# Autodesk Inventor assembly: 3d_Welding_Tooling - Lathe carriage
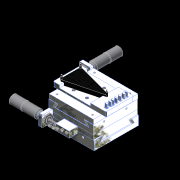
[picture p0: Inventor's stored thumbnail of the model, 180x180]
Saved by Autodesk Inventor 2018.3 (Build 223284000, 284)
## iProperties
Created: 2026-02-27
Part Number: 3d_Welding_Tooling - Lathe carriage
Document SubType Name: Assembly
Designer: aca6
Author: aca6
## Documents named in this file (19)
- C:\Users\aca6\git\LM\items\hw_LM\variants\items\Welding Tooling\3d\3d_Welding_Tooling - Lathe carriage.iam
- C:\Users\aca6\git\LM\items\hw_LM\variants\items\Welding Tooling\3d\3d_Welding_Tooling - Adapter.ipt
- C:\Users\aca6\git\LM\items\hw_LM\variants\items\Welding Tooling\3d\3d_Welding_Tooling -  Guide Pin.ipt
- C:\Users\aca6\git\LM\items\hw_LM\variants\items\Welding Tooling\3d\3d_Welding_Tooling - Top Adapter.ipt
- C:\Users\aca6\git\LM\items\hw_LM\variants\items\Welding Tooling\3d\3d_Welding_Tooling - Moving base.ipt
- C:\Users\aca6\git\LM\items\hw_LM\variants\items\Welding Tooling\3d\3d_Welding_Tooling - Fixed base.ipt
- C:\Users\aca6\git\LM\items\hw_LM\variants\items\Welding Tooling\3d\3d_Welding_Tooling - Acetal Stick.ipt
- C:\Users\aca6\git\LM\items\hw_LM\variants\items\Welding Tooling\3d\3d_Welding_Tooling - Upper fixed base.ipt
- C:\Users\aca6\git\LM\items\hw_LM\variants\items\Welding Tooling\3d\3d_Welding_Tooling - Upper moving base.ipt
- C:\Users\aca6\git\LM\items\_accesories\Tornilleria\Tornillos\3d_DIN 7991\3d\A4 Black Inox\DIN 7991 - M3x14 Black INOX.ipt
- C:\Users\aca6\git\LM\items\_accesories\Tornilleria\Tornillos\3d_DIN 7991\3d\A4 Black Inox\DIN 7991 - M3x12 Black INOX.ipt
- C:\Users\aca6\git\LM\items\hw_LM\variants\items\Welding Tooling\3d\3d_Welding_Tooling -  Micrometer Nut.ipt
- C:\Users\aca6\git\LM\items\hw_LM\variants\items\Welding Tooling\3d\3d_Welding_Tooling -  Micrometer.ipt
- C:\Users\aca6\git\LM\items\hw_LM\variants\items\Welding Tooling\3d\3d_Welding_Tooling - Fixed Block.ipt
- C:\Users\aca6\git\LM\items\hw_LM\variants\items\Welding Tooling\3d\3d_Welding_Tooling -  Moving Block.ipt
- C:\Users\aca6\git\LM\items\_accesories\Tornilleria\Tornillos\3d_Accu Group\3d\Prisionero nylon M4x7 REF SSN-M4-7.ipt
- C:\Users\aca6\git\LM\items\_accesories\Tornilleria\Tornillos\3d_DIN 912\3d\A4 Inox\DIN 912 - M3 x 0,5 x 8 -  INOX.ipt
- C:\Users\aca6\git\LM\items\_accesories\Tornilleria\Tornillos\3d_DIN 912\3d\A4 Inox\DIN 912 - M3 x 0,5 x 30 -  INOX.ipt
- C:\Users\aca6\git\LM\items\_accesories\Tornilleria\Tornillos\3d_DIN 912\3d\A4 Inox\DIN 912 - M3 x 0,5 x 10 -  INOX.ipt
## Components (51 placed, 18 different names)
1. 3d_Welding_Tooling - Adapter:1
2. 3d_Welding_Tooling -  Guide Pin:1
3. 3d_Welding_Tooling -  Guide Pin:2
4. 3d_Welding_Tooling -  Guide Pin:3
5. 3d_Welding_Tooling - Top Adapter:1
6. 3d_Welding_Tooling - Moving base:1
7. 3d_Welding_Tooling - Fixed base:1
8. 3d_Welding_Tooling - Acetal Stick:1
9. 3d_Welding_Tooling - Acetal Stick:2
10. 3d_Welding_Tooling - Upper fixed base:1
11. 3d_Welding_Tooling - Acetal Stick:3
12. 3d_Welding_Tooling - Acetal Stick:4
13. 3d_Welding_Tooling - Upper moving base:1
14. DIN 7991 - M3x14 Black INOX:1
15. DIN 7991 - M3x14 Black INOX:2
16. DIN 7991 - M3x14 Black INOX:3
17. DIN 7991 - M3x14 Black INOX:4
18. DIN 7991 - M3x12 Black INOX:1
19. DIN 7991 - M3x12 Black INOX:2
20. DIN 7991 - M3x12 Black INOX:3
21. DIN 7991 - M3x12 Black INOX:4
22. 3d_Welding_Tooling -  Micrometer Nut:1
23. 3d_Welding_Tooling -  Micrometer:1
24. 3d_Welding_Tooling -  Micrometer Nut:2
25. 3d_Welding_Tooling - Fixed Block:1
26. 3d_Welding_Tooling -  Moving Block:1
27. Prisionero nylon M4x7 REF SSN-M4-7:1
28. Prisionero nylon M4x7 REF SSN-M4-7:2
29. Prisionero nylon M4x7 REF SSN-M4-7:3
30. Prisionero nylon M4x7 REF SSN-M4-7:4
31. 3d_Welding_Tooling - Fixed Block:2
32. 3d_Welding_Tooling -  Micrometer:2
33. 3d_Welding_Tooling -  Moving Block:2
34. Prisionero nylon M4x7 REF SSN-M4-7:5
35. Prisionero nylon M4x7 REF SSN-M4-7:6
36. Prisionero nylon M4x7 REF SSN-M4-7:7
37. Prisionero nylon M4x7 REF SSN-M4-7:8
38. Prisionero nylon M4x7 REF SSN-M4-7:9
39. Prisionero nylon M4x7 REF SSN-M4-7:10
40. Prisionero nylon M4x7 REF SSN-M4-7:11
41. Prisionero nylon M4x7 REF SSN-M4-7:12
42. DIN 912 - M3 x 0,5 x 8 -  INOX:1
43. DIN 912 - M3 x 0,5 x 8 -  INOX:2
44. DIN 912 - M3 x 0,5 x 30 -  INOX:1
45. DIN 912 - M3 x 0,5 x 30 -  INOX:2
46. DIN 912 - M3 x 0,5 x 30 -  INOX:3
47. DIN 912 - M3 x 0,5 x 30 -  INOX:4
48. DIN 912 - M3 x 0,5 x 10 -  INOX:1
49. DIN 912 - M3 x 0,5 x 10 -  INOX:2
50. DIN 912 - M3 x 0,5 x 10 -  INOX:3
51. DIN 912 - M3 x 0,5 x 10 -  INOX:4
## Relationships (115: Mate 79, Flush 28, Tangent 8)
- [Mate]: 3d_Welding_Tooling - Adapter:1 ↔ 3d_Welding_Tooling -  Guide Pin:1
- [Mate]: 3d_Welding_Tooling - Adapter:1 ↔ 3d_Welding_Tooling -  Guide Pin:2
- [Mate]: 3d_Welding_Tooling - Adapter:1 ↔ 3d_Welding_Tooling -  Guide Pin:3
- [Mate]: 3d_Welding_Tooling - Adapter:1 ↔ 3d_Welding_Tooling -  Guide Pin:2
- [Mate]: 3d_Welding_Tooling - Adapter:1 ↔ 3d_Welding_Tooling -  Guide Pin:1
- [Mate]: 3d_Welding_Tooling - Adapter:1 ↔ 3d_Welding_Tooling -  Guide Pin:2
- [Mate]: 3d_Welding_Tooling - Adapter:1 ↔ 3d_Welding_Tooling -  Guide Pin:1
- [Mate]: 3d_Welding_Tooling - Adapter:1 ↔ 3d_Welding_Tooling -  Guide Pin:3
- [Flush]: 3d_Welding_Tooling - Adapter:1 ↔ 3d_Welding_Tooling - Top Adapter:1
- [Mate]: 3d_Welding_Tooling -  Guide Pin:2 ↔ 3d_Welding_Tooling - Top Adapter:1
- [Mate]: 3d_Welding_Tooling -  Guide Pin:1 ↔ 3d_Welding_Tooling - Top Adapter:1
- [Mate]: 3d_Welding_Tooling - Moving base:1 ↔ 3d_Welding_Tooling - Fixed base:1
- [Flush]: 3d_Welding_Tooling - Moving base:1 ↔ 3d_Welding_Tooling - Fixed base:1
- [Mate]: 3d_Welding_Tooling - Moving base:1 ↔ 3d_Welding_Tooling - Acetal Stick:1
- [Mate]: 3d_Welding_Tooling - Moving base:1 ↔ 3d_Welding_Tooling - Acetal Stick:1
- [Mate]: 3d_Welding_Tooling - Fixed base:1 ↔ 3d_Welding_Tooling - Acetal Stick:2
- [Mate]: 3d_Welding_Tooling - Fixed base:1 ↔ 3d_Welding_Tooling - Acetal Stick:2
- [Flush]: 3d_Welding_Tooling - Fixed base:1 ↔ 3d_Welding_Tooling - Acetal Stick:1
- [Flush]: 3d_Welding_Tooling - Fixed base:1 ↔ 3d_Welding_Tooling - Acetal Stick:2
- [Mate]: 3d_Welding_Tooling - Moving base:1 ↔ 3d_Welding_Tooling - Upper fixed base:1
- [Mate]: 3d_Welding_Tooling - Moving base:1 ↔ 3d_Welding_Tooling - Upper fixed base:1
- [Mate]: 3d_Welding_Tooling - Moving base:1 ↔ 3d_Welding_Tooling - Upper fixed base:1
- [Mate]: 3d_Welding_Tooling - Upper fixed base:1 ↔ 3d_Welding_Tooling - Acetal Stick:3
- [Mate]: 3d_Welding_Tooling - Upper fixed base:1 ↔ 3d_Welding_Tooling - Acetal Stick:3
- [Mate]: 3d_Welding_Tooling - Upper fixed base:1 ↔ 3d_Welding_Tooling - Acetal Stick:4
- [Mate]: 3d_Welding_Tooling - Upper fixed base:1 ↔ 3d_Welding_Tooling - Acetal Stick:4
- [Flush]: 3d_Welding_Tooling - Upper fixed base:1 ↔ 3d_Welding_Tooling - Acetal Stick:4
- [Flush]: 3d_Welding_Tooling - Upper fixed base:1 ↔ 3d_Welding_Tooling - Acetal Stick:3
- [Mate]: 3d_Welding_Tooling - Upper fixed base:1 ↔ 3d_Welding_Tooling - Upper moving base:1
- [Mate]: 3d_Welding_Tooling - Acetal Stick:4 ↔ 3d_Welding_Tooling - Upper moving base:1
- [Mate]: 3d_Welding_Tooling - Upper fixed base:1 ↔ DIN 7991 - M3x14 Black INOX:3
- [Mate]: 3d_Welding_Tooling - Upper fixed base:1 ↔ DIN 7991 - M3x14 Black INOX:4
- [Mate]: 3d_Welding_Tooling - Upper fixed base:1 ↔ DIN 7991 - M3x14 Black INOX:1
- [Mate]: 3d_Welding_Tooling - Upper fixed base:1 ↔ DIN 7991 - M3x14 Black INOX:2
- [Tangent]: 3d_Welding_Tooling - Upper fixed base:1 ↔ DIN 7991 - M3x14 Black INOX:4
- [Tangent]: 3d_Welding_Tooling - Upper fixed base:1 ↔ DIN 7991 - M3x14 Black INOX:2
- [Tangent]: 3d_Welding_Tooling - Upper fixed base:1 ↔ DIN 7991 - M3x14 Black INOX:1
- [Tangent]: 3d_Welding_Tooling - Upper fixed base:1 ↔ DIN 7991 - M3x14 Black INOX:3
- [Mate]: 3d_Welding_Tooling - Adapter:1 ↔ 3d_Welding_Tooling - Upper moving base:1
- [Flush] (18.75 mm): 3d_Welding_Tooling - Adapter:1 ↔ 3d_Welding_Tooling - Upper moving base:1
- [Flush] (-9.684 mm): 3d_Welding_Tooling - Adapter:1 ↔ 3d_Welding_Tooling - Upper moving base:1
- [Mate]: 3d_Welding_Tooling - Adapter:1 ↔ DIN 7991 - M3x12 Black INOX:4
- [Mate]: 3d_Welding_Tooling - Adapter:1 ↔ DIN 7991 - M3x12 Black INOX:1
- [Mate]: 3d_Welding_Tooling - Adapter:1 ↔ DIN 7991 - M3x12 Black INOX:3
- [Mate]: 3d_Welding_Tooling - Adapter:1 ↔ DIN 7991 - M3x12 Black INOX:2
- [Tangent]: 3d_Welding_Tooling - Adapter:1 ↔ DIN 7991 - M3x12 Black INOX:3
- [Tangent]: 3d_Welding_Tooling - Adapter:1 ↔ DIN 7991 - M3x12 Black INOX:2
- [Tangent]: 3d_Welding_Tooling - Adapter:1 ↔ DIN 7991 - M3x12 Black INOX:4
- [Tangent]: 3d_Welding_Tooling - Adapter:1 ↔ DIN 7991 - M3x12 Black INOX:1
- [Mate]: 3d_Welding_Tooling -  Micrometer:1 ↔ 3d_Welding_Tooling - Fixed Block:1
- [Mate]: 3d_Welding_Tooling -  Micrometer:1 ↔ 3d_Welding_Tooling - Fixed Block:1
- [Mate]: 3d_Welding_Tooling -  Micrometer:1 ↔ 3d_Welding_Tooling -  Micrometer Nut:2
- [Mate]: 3d_Welding_Tooling -  Micrometer Nut:2 ↔ 3d_Welding_Tooling - Fixed Block:1
- [Mate]: 3d_Welding_Tooling - Upper fixed base:1 ↔ 3d_Welding_Tooling - Fixed Block:1
- [Flush]: 3d_Welding_Tooling - Upper fixed base:1 ↔ 3d_Welding_Tooling - Fixed Block:1
- [Mate]: 3d_Welding_Tooling - Upper moving base:1 ↔ 3d_Welding_Tooling -  Moving Block:1
- [Flush]: 3d_Welding_Tooling - Upper fixed base:1 ↔ 3d_Welding_Tooling - Upper moving base:1
- [Flush]: 3d_Welding_Tooling - Moving base:1 ↔ 3d_Welding_Tooling - Fixed base:1
- [Mate]: 3d_Welding_Tooling - Upper fixed base:1 ↔ Prisionero nylon M4x7 REF SSN-M4-7:1
- [Mate]: 3d_Welding_Tooling - Fixed base:1 ↔ Prisionero nylon M4x7 REF SSN-M4-7:2
- [Mate]: 3d_Welding_Tooling - Upper fixed base:1 ↔ Prisionero nylon M4x7 REF SSN-M4-7:4
- [Mate]: 3d_Welding_Tooling - Fixed base:1 ↔ Prisionero nylon M4x7 REF SSN-M4-7:3
- [Flush]: 3d_Welding_Tooling - Fixed base:1 ↔ Prisionero nylon M4x7 REF SSN-M4-7:3
- [Flush]: 3d_Welding_Tooling - Fixed base:1 ↔ Prisionero nylon M4x7 REF SSN-M4-7:2
- [Flush]: 3d_Welding_Tooling - Upper fixed base:1 ↔ Prisionero nylon M4x7 REF SSN-M4-7:1
- [Flush]: 3d_Welding_Tooling - Upper fixed base:1 ↔ Prisionero nylon M4x7 REF SSN-M4-7:4
- [Flush]: 3d_Welding_Tooling - Upper fixed base:1 ↔ 3d_Welding_Tooling - Fixed Block:1
- [Mate]: 3d_Welding_Tooling - Fixed base:1 ↔ 3d_Welding_Tooling - Fixed Block:2
- [Flush]: 3d_Welding_Tooling - Fixed base:1 ↔ 3d_Welding_Tooling - Fixed Block:2
- [Flush]: 3d_Welding_Tooling - Fixed base:1 ↔ 3d_Welding_Tooling - Fixed Block:2
- [Mate]: 3d_Welding_Tooling - Fixed Block:2 ↔ 3d_Welding_Tooling -  Micrometer:2
- [Mate]: 3d_Welding_Tooling - Fixed Block:2 ↔ 3d_Welding_Tooling -  Micrometer:2
- [Mate]: 3d_Welding_Tooling -  Micrometer Nut:1 ↔ 3d_Welding_Tooling -  Micrometer:2
- [Mate]: 3d_Welding_Tooling -  Micrometer Nut:1 ↔ 3d_Welding_Tooling - Fixed Block:2
- [Mate]: 3d_Welding_Tooling - Moving base:1 ↔ 3d_Welding_Tooling -  Moving Block:2
- [Mate]: 3d_Welding_Tooling - Upper moving base:1 ↔ Prisionero nylon M4x7 REF SSN-M4-7:5
- [Mate]: 3d_Welding_Tooling - Upper moving base:1 ↔ Prisionero nylon M4x7 REF SSN-M4-7:8
- [Mate]: 3d_Welding_Tooling - Upper moving base:1 ↔ Prisionero nylon M4x7 REF SSN-M4-7:7
- [Mate]: 3d_Welding_Tooling - Upper moving base:1 ↔ Prisionero nylon M4x7 REF SSN-M4-7:6
- [Flush]: 3d_Welding_Tooling - Upper moving base:1 ↔ Prisionero nylon M4x7 REF SSN-M4-7:6
- [Flush]: 3d_Welding_Tooling - Upper moving base:1 ↔ Prisionero nylon M4x7 REF SSN-M4-7:5
- [Flush]: 3d_Welding_Tooling - Upper moving base:1 ↔ Prisionero nylon M4x7 REF SSN-M4-7:7
- [Flush]: 3d_Welding_Tooling - Upper moving base:1 ↔ Prisionero nylon M4x7 REF SSN-M4-7:8
- [Mate]: 3d_Welding_Tooling - Fixed base:1 ↔ Prisionero nylon M4x7 REF SSN-M4-7:9
- [Flush]: 3d_Welding_Tooling - Fixed base:1 ↔ Prisionero nylon M4x7 REF SSN-M4-7:9
- [Mate]: 3d_Welding_Tooling - Fixed base:1 ↔ Prisionero nylon M4x7 REF SSN-M4-7:10
- [Flush]: 3d_Welding_Tooling - Fixed base:1 ↔ Prisionero nylon M4x7 REF SSN-M4-7:10
- [Mate]: 3d_Welding_Tooling - Upper fixed base:1 ↔ Prisionero nylon M4x7 REF SSN-M4-7:11
- [Flush]: 3d_Welding_Tooling - Upper fixed base:1 ↔ Prisionero nylon M4x7 REF SSN-M4-7:11
- [Mate]: 3d_Welding_Tooling - Upper fixed base:1 ↔ Prisionero nylon M4x7 REF SSN-M4-7:12
- [Flush]: 3d_Welding_Tooling - Upper fixed base:1 ↔ Prisionero nylon M4x7 REF SSN-M4-7:12
- [Mate]: 3d_Welding_Tooling -  Moving Block:2 ↔ DIN 912 - M3 x 0,5 x 8 -  INOX:2
- [Mate]: 3d_Welding_Tooling -  Moving Block:2 ↔ DIN 912 - M3 x 0,5 x 8 -  INOX:2
- [Mate]: 3d_Welding_Tooling -  Moving Block:1 ↔ DIN 912 - M3 x 0,5 x 8 -  INOX:1
- [Mate]: 3d_Welding_Tooling -  Moving Block:1 ↔ DIN 912 - M3 x 0,5 x 8 -  INOX:1
- [Mate]: 3d_Welding_Tooling -  Micrometer:2 ↔ 3d_Welding_Tooling -  Moving Block:2
- [Mate]: 3d_Welding_Tooling -  Micrometer:1 ↔ 3d_Welding_Tooling -  Moving Block:1
- [Flush] (50 mm): 3d_Welding_Tooling - Upper moving base:1 ↔ 3d_Welding_Tooling -  Moving Block:1
- [Flush] (50 mm): 3d_Welding_Tooling - Moving base:1 ↔ 3d_Welding_Tooling -  Moving Block:2
- [Mate]: 3d_Welding_Tooling -  Moving Block:2 ↔ DIN 912 - M3 x 0,5 x 30 -  INOX:2
- [Mate]: 3d_Welding_Tooling -  Moving Block:2 ↔ DIN 912 - M3 x 0,5 x 30 -  INOX:1
- [Mate]: 3d_Welding_Tooling -  Moving Block:2 ↔ DIN 912 - M3 x 0,5 x 30 -  INOX:2
- [Mate]: 3d_Welding_Tooling -  Moving Block:2 ↔ DIN 912 - M3 x 0,5 x 30 -  INOX:1
- [Mate]: 3d_Welding_Tooling -  Moving Block:1 ↔ DIN 912 - M3 x 0,5 x 30 -  INOX:3
- [Mate]: 3d_Welding_Tooling -  Moving Block:1 ↔ DIN 912 - M3 x 0,5 x 30 -  INOX:4
- [Mate]: 3d_Welding_Tooling -  Moving Block:1 ↔ DIN 912 - M3 x 0,5 x 30 -  INOX:4
- [Mate]: 3d_Welding_Tooling -  Moving Block:1 ↔ DIN 912 - M3 x 0,5 x 30 -  INOX:3
- [Mate]: 3d_Welding_Tooling - Fixed Block:1 ↔ DIN 912 - M3 x 0,5 x 10 -  INOX:2
- [Mate]: 3d_Welding_Tooling - Fixed Block:1 ↔ DIN 912 - M3 x 0,5 x 10 -  INOX:1
- [Mate]: 3d_Welding_Tooling - Fixed Block:1 ↔ DIN 912 - M3 x 0,5 x 10 -  INOX:1
- [Mate]: 3d_Welding_Tooling - Fixed Block:1 ↔ DIN 912 - M3 x 0,5 x 10 -  INOX:2
- [Mate]: 3d_Welding_Tooling - Fixed Block:2 ↔ DIN 912 - M3 x 0,5 x 10 -  INOX:4
- [Mate]: 3d_Welding_Tooling - Fixed Block:2 ↔ DIN 912 - M3 x 0,5 x 10 -  INOX:3
- [Mate]: 3d_Welding_Tooling - Fixed Block:2 ↔ DIN 912 - M3 x 0,5 x 10 -  INOX:3
- [Mate]: 3d_Welding_Tooling - Fixed Block:2 ↔ DIN 912 - M3 x 0,5 x 10 -  INOX:4
## Named parameters: d236_d199 = 0 mm, d237_d201 = 0 mm, d238_d203 = 0 mm, d239_d204 = 0 mm, d86_d91 = 0 mm, d87_d92 = 0 mm, d88_d93 = 0 mm, d89_d95 = 0 mm, d90_d96 = 0 mm, d91_d97 = 0 mm, d92_d98 = 0 mm, d93_d99 = 0 mm
